# Autodesk Inventor assembly: Цепной привод2_MIR_MIR
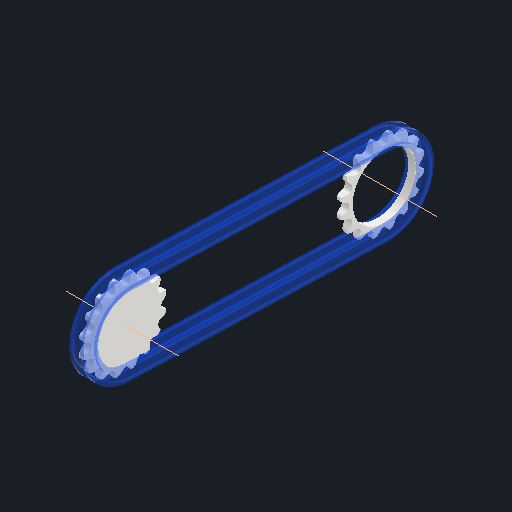
[picture p0: Inventor's stored thumbnail of the model, 512x512]
Saved by Autodesk Inventor 2025 (Build 290162000, 162)
## iProperties
Created: 2024-09-18
Part Number: Цепной привод2_MIR_MIR
Document SubType Name: Assembly
Designer: GameHD
Author: GameHD
## Documents named in this file (4)
- C:\Users\GameHD\Desktop\КАРКАС с цепями 2\цепь\Мастер проектирования\Цепной привод2_MIR_MIR.iam
- C:\Users\GameHD\Desktop\КАРКАС с цепями 2\цепь\Мастер проектирования\Цепь роликовая2_MIR_MIR.ipt
- C:\Users\GameHD\Desktop\КАРКАС с цепями 2\цепь\Мастер проектирования\Звездочка роликовой цепи12_MIR_MIR.ipt
- C:\Users\GameHD\Desktop\КАРКАС с цепями 2\цепь\Мастер проектирования\Звездочка роликовой цепи22_MIR_MIR.ipt
## Components (3 placed, 3 different names)
1. Цепь роликовая2_MIR_MIR:1 — Заподлицо:1, Совмещение:1, Совмещение:2, Заподлицо:2, Совмещение:3, Совмещение:4
2. Звездочка роликовой цепи12_MIR_MIR:1 — Заподлицо:1, Совмещение:1, Совмещение:2, ЗубчПер:1
3. Звездочка роликовой цепи22_MIR_MIR:1 — Заподлицо:2, Совмещение:3, Совмещение:4, ЗубчПер:1
## Relationships (7: Mate 4, Flush 2, RelateRotation 1)
- Заподлицо:1 [Flush]: Цепь роликовая2_MIR_MIR:1 ↔ Звездочка роликовой цепи12_MIR_MIR:1
- Совмещение:1 [Mate]: Цепь роликовая2_MIR_MIR:1 ↔ Звездочка роликовой цепи12_MIR_MIR:1
- Совмещение:2 [Mate]: Цепь роликовая2_MIR_MIR:1 ↔ Звездочка роликовой цепи12_MIR_MIR:1
- Заподлицо:2 [Flush]: Цепь роликовая2_MIR_MIR:1 ↔ Звездочка роликовой цепи22_MIR_MIR:1
- Совмещение:3 [Mate]: Цепь роликовая2_MIR_MIR:1 ↔ Звездочка роликовой цепи22_MIR_MIR:1
- Совмещение:4 [Mate]: Цепь роликовая2_MIR_MIR:1 ↔ Звездочка роликовой цепи22_MIR_MIR:1
- ЗубчПер:1 [RelateRotation] (1 ul): Звездочка роликовой цепи12_MIR_MIR:1 ↔ Звездочка роликовой цепи22_MIR_MIR:1
